# Autodesk Inventor assembly: RPI
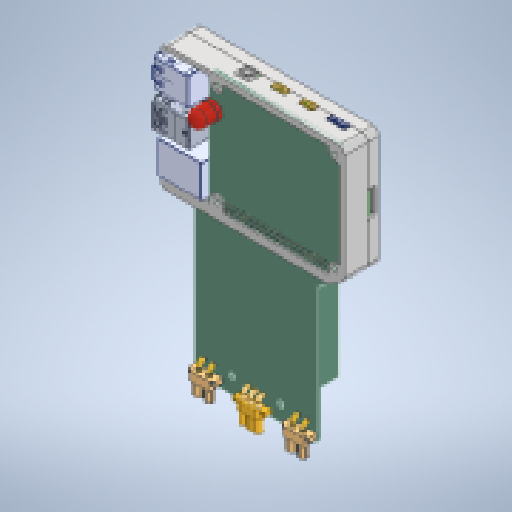
[picture p0: Inventor's stored thumbnail of the model, 512x512]
Saved by Autodesk Inventor 2023.4 (Build 274418000, 418)
## iProperties
Created: 2024-09-15
Part Number: RPI
Document SubType Name: Assembly
Designer: komputer
Author: komputer
## Documents named in this file (5)
- E:\PROJECTS_REPOS\Robal-2.0\mechanics\RPI.iam
- E:\PROJECTS_REPOS\Robal-2.0\mechanics\step\robal_rpi_ioBoard\robal_rpi_ioBoard.ipt
- E:\PROJECTS_REPOS\Robal-2.0\mechanics\rpi_wspornik.ipt
- E:\PROJECTS_REPOS\Robal-2.0\mechanics\podstawa_rpi_1.ipt
- E:\PROJECTS_REPOS\Robal-2.0\mechanics\podstawa_rpi_board_2.ipt
## Components (4 placed, 4 different names)
1. robal_rpi_ioBoard:1 — Flush:1, Flush:2
2. rpi_wspornik:1 — Flush:1, Flush:3
3. podstawa_rpi_1:1 — Flush:2
4. podstawa_rpi_board_2:1 — Flush:3
## Relationships (3: Flush 3)
- Flush:1: robal_rpi_ioBoard:1 ↔ rpi_wspornik:1
- Flush:2: robal_rpi_ioBoard:1 ↔ podstawa_rpi_1:1
- Flush:3: rpi_wspornik:1 ↔ podstawa_rpi_board_2:1
